# Autodesk Inventor assembly: ISISpace 1U Frame
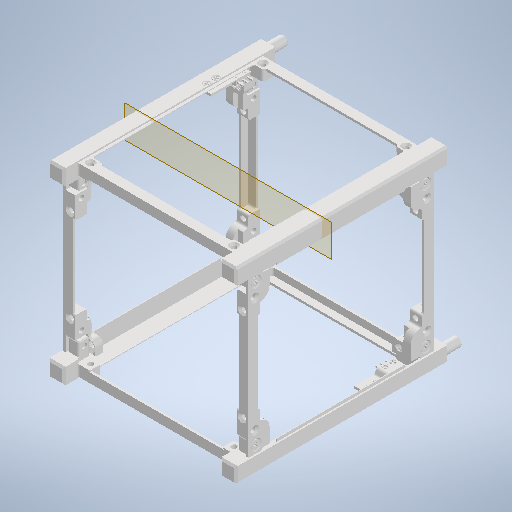
[picture p0: Inventor's stored thumbnail of the model, 512x512]
Saved by Autodesk Inventor 2025 (Build 290162000, 162)
## iProperties
Created: 2011-03-02
Part Number: ISISpace 1U Frame
Document SubType Name: Assembly
Designer: Andrew Robinson
Engineer: GAR
Sending System: PRO/ENGINEER BY PARAMETRIC TECHNOLOGY CORPORATION, 2003250
Preprocessor: PRO/ENGINEER BY PARAMETRIC TECHNOLOGY CORPORATION, 2003250
Title: ISISpace 1U Frame
Revision Number: LAST_VERSION
## Documents named in this file (3)
- C:\Users\arobi\Documents\Repos\fox-plus\mechanical\AssemblyModels\ISIS CubeSat STS PC104 Skeleton.iam
- C:\Users\arobi\Documents\Repos\fox-plus\mechanical\AssemblyModels\INTEGRATED_SIDE_FRAME_007B_ASM.iam
- C:\Users\arobi\Documents\Repos\fox-plus\mechanical\AssemblyModels\REVE_02-1_ASSEMBLY_RIB_CDEF_ASM.iam
## Components (3 placed, 3 different names)
1. INTEGRATED_SIDE_FRAME_007B_ASM_22 [sub-assembly]
2. INTEGRATED_SIDE_FRAME_007B_ASM_23 [sub-assembly] — Mate:1, Angle:1
3. REVE_02-1_ASSEMBLY_RIB_CDEF_ASM_32 [sub-assembly]
## Relationships (3: Mate 1, Angle 1, Flush 1)
- Mate:1: INTEGRATED_SIDE_FRAME_007B_ASM_23
- Angle:1 (0 deg): INTEGRATED_SIDE_FRAME_007B_ASM_23
- Flush:1 (-45 mm)
